# Autodesk Inventor assembly: Ensamble caja
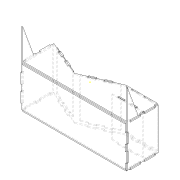
[picture p0: Inventor's stored thumbnail of the model, 180x180]
Saved by Autodesk Inventor 2022 (Build 260153000, 153)
## iProperties
Created: 2022-06-06
Part Number: Ensamble caja
Document SubType Name: Assembly
Designer: ADMIN
Author: ADMIN
## Documents named in this file (7)
- G:\Unidades compartidas\TP1 2022-I\no c\Ensamble caja.iam
- G:\Unidades compartidas\TP1 2022-I\no c\Modelo base.ipt
- G:\Unidades compartidas\TP1 2022-I\no c\Lateral.ipt
- G:\Unidades compartidas\TP1 2022-I\no c\Frontal.ipt
- G:\Unidades compartidas\TP1 2022-I\no c\Fondo.ipt
- G:\Unidades compartidas\TP1 2022-I\no c\Piso.ipt
- G:\Unidades compartidas\TP1 2022-I\no c\Top 1.ipt
## Components (10 placed, 6 different names)
1. Modelo base:1 — Flush:1, Flush:2, Flush:3, Flush:4, Mate:1, Flush:5, Flush:6, Flush:7, Flush:8
2. Lateral:1 — Flush:1
3. Frontal:1 — Flush:2, Flush:3, Mate:2, Mate:3, Mate:4, Mate:5, Mate:6, Mate:7
4. Lateral:2 — Flush:4, Flush:5, Mate:1
5. Fondo:1 — Flush:6
6. Piso:1 — Flush:7
7. Top 1:1 — Flush:8
8. Top 1:2 — Mate:2, Mate:3
9. Top 1:3 — Mate:4, Mate:5, Flush:9
10. Top 1:4 — Mate:6, Flush:9, Mate:7
## Relationships (16: Flush 9, Mate 7)
- Flush:1: Modelo base:1 ↔ Lateral:1
- Flush:2: Modelo base:1 ↔ Frontal:1
- Flush:3: Modelo base:1 ↔ Frontal:1
- Flush:4: Modelo base:1 ↔ Lateral:2
- Flush:5: Modelo base:1 ↔ Lateral:2
- Mate:1: Modelo base:1 ↔ Lateral:2
- Flush:6: Modelo base:1 ↔ Fondo:1
- Flush:7: Modelo base:1 ↔ Piso:1
- Flush:8: Modelo base:1 ↔ Top 1:1
- Mate:2: Frontal:1 ↔ Top 1:2
- Mate:3: Frontal:1 ↔ Top 1:2
- Mate:4: Frontal:1 ↔ Top 1:3
- Mate:5: Frontal:1 ↔ Top 1:3
- Mate:6: Frontal:1 ↔ Top 1:4
- Flush:9: Top 1:3 ↔ Top 1:4
- Mate:7: Frontal:1 ↔ Top 1:4
